# Autodesk Inventor assembly: Application_Incubator_Microscope_v2
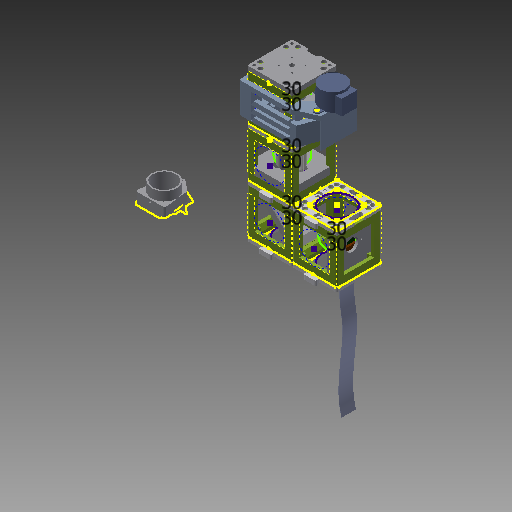
[picture p0: Inventor's stored thumbnail of the model, 512x512]
Saved by Autodesk Inventor 2019 (Build 230136000, 136)
## iProperties
Created: 2019-07-16
Part Number: Application_Incubator_Microscope_v2
Document SubType Name: Assembly
Designer: marsikovabarbora
Author: marsikovabarbora
## Documents named in this file (5)
- C:\Users\marsikovabarbora\Dropbox\UC2\02_CAD\INVENTOR\uc2_v3\Application_Incubator_Microscope_v2.iam
- C:\Users\marsikovabarbora\Dropbox\UC2\02_CAD\INVENTOR\uc2_v3\Assembly_Cube_Mirror_30x30_v3.iam
- C:\Users\marsikovabarbora\Dropbox\UC2\02_CAD\INVENTOR\uc2_v3\Assembly_Cube_RaspiCam_v3.iam
- C:\Users\marsikovabarbora\Dropbox\UC2\02_CAD\INVENTOR\uc2_v3\10_Base_puzzle_v3.ipt
- C:\Users\marsikovabarbora\Dropbox\UC2\02_CAD\INVENTOR\uc2_v3\Assembly_Cube_Z-Focus_Sample_v3.iam
## Components (7 placed, 4 different names)
1. Assembly_Cube_Mirror_30x30_v3:1 [sub-assembly] — Mate:11
2. Assembly_Cube_RaspiCam_v3:1 [sub-assembly] — Passend:3, Winkel:1, Passend:4, Passend:7
3. Assembly_Cube_Z-Focus_Sample_v3:1 [sub-assembly] — Mate:10, Angle:3
4. 10_Base_puzzle_v3:1 — Passend:7
5. 10_Base_puzzle_v3:3 — Mate:10, Angle:3
6. 10_Base_puzzle_v3:2 — Passend:3, Winkel:1, Passend:4
7. 10_Base_puzzle_v3:4 — Passend:1, Fluchtend:1, Passend:2, Mate:11
## Component patterns: (2 elements, first: 10_Base_puzzle_v3:1), (2 elements, first: 10_Base_puzzle_v3:2)
## Relationships (10: Mate 7, Angle 2, Flush 1)
- Passend:1 [Mate]: 10_Base_puzzle_v3:4
- Fluchtend:1 [Flush]: 10_Base_puzzle_v3:4
- Passend:2 [Mate]: 10_Base_puzzle_v3:4
- Passend:3 [Mate]: Assembly_Cube_RaspiCam_v3:1 ↔ 10_Base_puzzle_v3:2
- Winkel:1 [Angle] (0 deg): Assembly_Cube_RaspiCam_v3:1 ↔ 10_Base_puzzle_v3:2
- Passend:4 [Mate]: Assembly_Cube_RaspiCam_v3:1 ↔ 10_Base_puzzle_v3:2
- Passend:7 [Mate]: Assembly_Cube_RaspiCam_v3:1 ↔ 10_Base_puzzle_v3:1
- Mate:10: Assembly_Cube_Z-Focus_Sample_v3:1 ↔ 10_Base_puzzle_v3:3
- Angle:3 (0 deg): Assembly_Cube_Z-Focus_Sample_v3:1 ↔ 10_Base_puzzle_v3:3
- Mate:11: Assembly_Cube_Mirror_30x30_v3:1 ↔ 10_Base_puzzle_v3:4
